# Autodesk Inventor assembly: Ground_Tracker
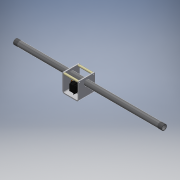
[picture p0: Inventor's stored thumbnail of the model, 180x180]
Saved by Autodesk Inventor 2018 (Build 220112000, 112)
## iProperties
Created: 2018-09-27
Part Number: Ground_Tracker
Document SubType Name: Assembly
Designer: Bradley
Author: Bradley
## Documents named in this file (7)
- C:\Users\Bradley\Documents\GitHub\CougSat1-Hardware\CougSat1-GroundStation\CADModel\Native\Ground_Tracker.iam
- C:\Users\Bradley\Documents\GitHub\CougSat1-Hardware\CougSat1-GroundStation\CADModel\Native\Ground_Tracker_TripodMount.ipt
- C:\Users\Bradley\Documents\GitHub\CougSat1-Hardware\CougSat1-GroundStation\CADModel\Native\Ground_Tracker_Bearing.ipt
- C:\Users\Bradley\Documents\GitHub\CougSat1-Hardware\CougSat1-GroundStation\CADModel\Native\Ground_Tracker_CrossTube.ipt
- C:\Users\Bradley\Documents\GitHub\Resources\ComponentModels\Hardware\Coupler_ServoHub.ipt
- C:\Users\Bradley\Documents\GitHub\Resources\ComponentModels\Electronics\Servo_Standard.ipt
- C:\Users\Bradley\Documents\GitHub\CougSat1-Hardware\CougSat1-GroundStation\CADModel\Native\Ground_Tracker_Spacer.ipt
## Components (8 placed, 6 different names)
1. Ground_Tracker_TripodMount:1 — Insert:1, Insert:2, Insert:3
2. Ground_Tracker_Bearing:1 — Insert:1, Mate:1, Flush:1, Mate:2, Insert:5, Insert:6
3. Ground_Tracker_CrossTube:1 — Mate:1, Flush:1
4. Coupler_ServoHub:1 — Insert:2, Insert:3, Insert:4
5. Servo_Standard:1 — Insert:4
6. Servo_Standard:2 — Mate:2
7. Ground_Tracker_Spacer:1 — Insert:5
8. Ground_Tracker_Spacer:2 — Insert:6
## Relationships (9: Insert 6, Mate 2, Flush 1)
- Insert:1: Ground_Tracker_TripodMount:1 ↔ Ground_Tracker_Bearing:1
- Mate:1: Ground_Tracker_Bearing:1 ↔ Ground_Tracker_CrossTube:1
- Flush:1 (70 mm): Ground_Tracker_Bearing:1 ↔ Ground_Tracker_CrossTube:1
- Insert:2: Ground_Tracker_TripodMount:1 ↔ Coupler_ServoHub:1
- Insert:3: Ground_Tracker_TripodMount:1 ↔ Coupler_ServoHub:1
- Insert:4: Coupler_ServoHub:1 ↔ Servo_Standard:1
- Mate:2 (10 mm): Ground_Tracker_Bearing:1 ↔ Servo_Standard:2
- Insert:5: Ground_Tracker_Bearing:1 ↔ Ground_Tracker_Spacer:1
- Insert:6: Ground_Tracker_Bearing:1 ↔ Ground_Tracker_Spacer:2
